# Autodesk Inventor assembly: updatedtestsectionassembly + Platform
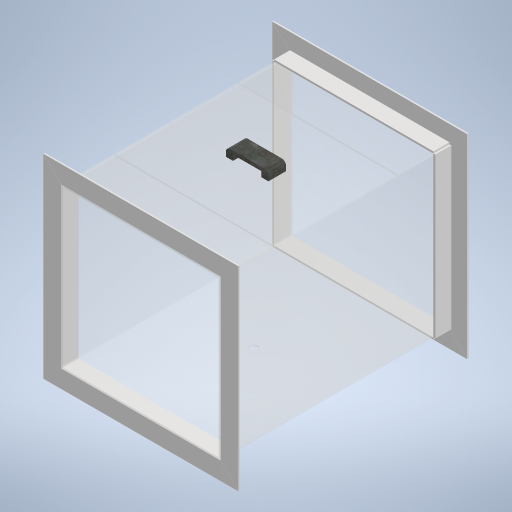
[picture p0: Inventor's stored thumbnail of the model, 512x512]
Saved by Autodesk Inventor 2023 (Build 270158000, 158)
## iProperties
Created: 2021-08-04
Part Number: updatedtestsectionassembly + Platform
Document SubType Name: Assembly
Designer: Caleb
Author: Caleb
## Documents named in this file (10)
- C:\Users\earls\Documents\stewart-platform\CAD\Wind tunnel\TEST SECTION\updatedtestsectionassembly + Platform.iam
- C:\Users\earls\Documents\stewart-platform\CAD\Wind tunnel\TEST SECTION\newbottom.ipt
- C:\Users\earls\Documents\stewart-platform\CAD\Wind tunnel\TEST SECTION\newsides.ipt
- C:\Users\earls\Documents\stewart-platform\CAD\Wind tunnel\TEST SECTION\new topsides.ipt
- C:\Users\earls\Documents\stewart-platform\CAD\Wind tunnel\TEST SECTION\newmiddle.ipt
- C:\Users\earls\Documents\stewart-platform\CAD\Wind tunnel\TEST SECTION\newsteelhandle.ipt
- C:\Users\earls\Documents\stewart-platform\CAD\Wind tunnel\TEST SECTION\angle1.ipt
- C:\Users\earls\Documents\stewart-platform\CAD\Wind tunnel\TEST SECTION\angle2.ipt
- C:\Users\earls\Documents\stewart-platform\CAD\Wind tunnel\TEST SECTION\angle3.ipt
- C:\Users\earls\Documents\stewart-platform\CAD\Wind tunnel\TEST SECTION\angle4.ipt
## Components (15 placed, 9 different names)
1. newbottom:1 — Mate:1, Mate:2, Mate:3, Mate:4, Mate:12, Mate:13, Mate:22, Mate:23
2. newsides:1 — Mate:3, Mate:4, Mate:5, Mate:18, Mate:24
3. newsides:2 — Mate:1, Mate:2, Mate:6, Mate:7, Mate:8, Mate:9, Mate:16, Mate:26
4. new topsides:1 — Mate:5, Mate:6, Mate:10, Mate:14, Mate:15, Mate:17
5. new topsides:2 — Mate:7, Mate:8, Mate:20, Mate:21, Mate:25
6. newmiddle:1 — Mate:9, Mate:10, Rigid:2
7. angle1:1 — Mate:12, Mate:13
8. angle2:1 — Mate:14, Mate:15, Mate:19
9. angle3:1 — Mate:16, Mate:17
10. angle4:1 — Mate:18, Mate:19
11. angle1:2 — Mate:20, Mate:21, Mate:27
12. angle2:2 — Mate:22, Mate:23
13. angle3:2 — Mate:24, Mate:25
14. angle4:2 — Mate:26, Mate:27
15. newsteelhandle:1 — Rigid:2
## Relationships (27: Mate 26, WeldJoint 1)
- Mate:1: newbottom:1 ↔ newsides:2
- Mate:2: newbottom:1 ↔ newsides:2
- Mate:3: newbottom:1 ↔ newsides:1
- Mate:4: newbottom:1 ↔ newsides:1
- Mate:5: newsides:1 ↔ new topsides:1
- Mate:6: newsides:2 ↔ new topsides:1
- Mate:7: newsides:2 ↔ new topsides:2
- Mate:8: newsides:2 ↔ new topsides:2
- Mate:9: newsides:2 ↔ newmiddle:1
- Mate:10: new topsides:1 ↔ newmiddle:1
- Mate:12: newbottom:1 ↔ angle1:1
- Mate:13: newbottom:1 ↔ angle1:1
- Mate:14: new topsides:1 ↔ angle2:1
- Mate:15: new topsides:1 ↔ angle2:1
- Mate:16: newsides:2 ↔ angle3:1
- Mate:17: new topsides:1 ↔ angle3:1
- Mate:18: newsides:1 ↔ angle4:1
- Mate:19: angle2:1 ↔ angle4:1
- Mate:20: new topsides:2 ↔ angle1:2
- Mate:21: new topsides:2 ↔ angle1:2
- Mate:22: newbottom:1 ↔ angle2:2
- Mate:23: newbottom:1 ↔ angle2:2
- Mate:24: newsides:1 ↔ angle3:2
- Mate:25: new topsides:2 ↔ angle3:2
- Mate:26: newsides:2 ↔ angle4:2
- Mate:27: angle1:2 ↔ angle4:2
- Rigid:2 [WeldJoint]: newmiddle:1 ↔ newsteelhandle:1
